# Autodesk Inventor assembly: Assembly2
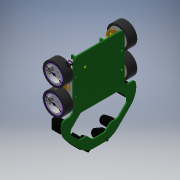
[picture p0: Inventor's stored thumbnail of the model, 180x180]
Saved by Autodesk Inventor 2016 (Build 200138000, 138)
## iProperties
Created: 2017-05-26
Part Number: Assembly2
Material: Ogólny
Document SubType Name: Assembly
Designer: Karol
Author: Karol
## Documents named in this file (32)
- D:\Git\MicromouseDixi\hardware\models\Dixi.iam
- D:\Git\MicromouseDixi\hardware\models\wheel.ipt
- D:\Git\MicromouseDixi\hardware\models\togh.ipt
- D:\Git\MicromouseDixi\hardware\models\bolt.ipt
- D:\Git\MicromouseDixi\hardware\models\magnet.ipt
- D:\Git\MicromouseDixi\hardware\models\mainpcb.ipt
- D:\Git\MicromouseDixi\hardware\models\motor.ipt
- D:\Git\MicromouseDixi\hardware\models\top_mount.ipt
- D:\Git\MicromouseDixi\hardware\models\XSM_0203_03_1.ipt
- D:\Git\MicromouseDixi\hardware\models\XFM_020406_03_233.ipt
- D:\Git\MicromouseDixi\hardware\models\enc_pcb.ipt
- D:\Git\MicromouseDixi\hardware\models\tyre.ipt
- D:\Git\MicromouseDixi\hardware\models\Dixi\Design Accelerator\Spur Gears4.iam
- D:\Git\MicromouseDixi\hardware\models\Dixi\Design Accelerator\Spur Gears3.iam
- D:\Git\MicromouseDixi\hardware\models\magnet_holder.ipt
- D:\Git\MicromouseDixi\hardware\models\tssop14.iam
- D:\Git\MicromouseDixi\hardware\models\led_mount.ipt
- D:\Git\MicromouseDixi\hardware\models\bolt_MIR.ipt
- D:\Git\MicromouseDixi\hardware\models\wheel_MIR.ipt
- D:\Git\MicromouseDixi\hardware\models\magnet_MIR.ipt
- D:\Git\MicromouseDixi\hardware\models\togh_MIR.ipt
- D:\Git\MicromouseDixi\hardware\models\motor_MIR.ipt
- D:\Git\MicromouseDixi\hardware\models\top_mount_MIR.ipt
- D:\Git\MicromouseDixi\hardware\models\XSM_0203_03_1_MIR.ipt
- D:\Git\MicromouseDixi\hardware\models\XFM_020406_03_233_MIR.ipt
- D:\Git\MicromouseDixi\hardware\models\enc_pcb_MIR.ipt
- D:\Git\MicromouseDixi\hardware\models\tyre_MIR.ipt
- D:\Git\MicromouseDixi\hardware\models\Dixi\Design Accelerator\Spur Gears4_MIR.iam
- D:\Git\MicromouseDixi\hardware\models\Dixi\Design Accelerator\Spur Gears3_MIR.iam
- D:\Git\MicromouseDixi\hardware\models\magnet_holder_MIR.ipt
- D:\Git\MicromouseDixi\hardware\models\tssop14_MIR.iam
- D:\Git\MicromouseDixi\hardware\models\led_mount_MIR.ipt
## Components (47 placed, 30 different names)
1. mainpcb:1 — Rotational:1, Rigid:47, Mate:1, Mate:2, Rigid:54
2. bolt:3 — Rigid:15, Rigid:45, Rotational:2
3. bolt:4 — Rigid:14, Rigid:46, Rigid:51, Rigid:52
4. wheel:3 — Rigid:15, Rigid:50
5. wheel:4 — Rigid:14, Rigid:49
6. magnet:4 — Rigid:53
7. togh:2 — Rigid:39, Rigid:40, Rigid:41, Rigid:44, Rotational:1, Rigid:47
8. motor:1 — Rigid:39, Rotational:3
9. top_mount:1 — Rigid:40
10. XSM_0203_03_1:1 — Rigid:42, Rigid:45
11. XFM_020406_03_233:1 — Rigid:41, Rigid:42
12. XSM_0203_03_1:2 — Rigid:46
13. XFM_020406_03_233:2 — Rigid:44
14. enc_pcb:1 — Planar:1, Rigid:54
15. tyre:1 — Rigid:49
16. tyre:2 — Rigid:50
17. Spur Gears:2 [sub-assembly] — Rigid:51
18. Spur Gears:7 [sub-assembly] — Rotational:2
19. Spur Gears:8 [sub-assembly] — Rotational:3
20. magnet_holder:1 — Rigid:52, Rigid:53
21. tssop14:1 [sub-assembly] — Planar:1
22. led_mount:1
23. led_mount:2
24. led_mount:3
25. bolt_MIR:1 — Rigid:55, Rigid:59, Rotational:4
26. bolt_MIR:2 — Rigid:56, Rigid:62, Rigid:67, Rigid:69
27. wheel_MIR:1 — Rigid:55, Rigid:66
28. wheel_MIR:2 — Rigid:56, Rigid:65
29. magnet_MIR:1 — Rigid:68
30. togh_MIR:1 — Rigid:57, Rigid:58, Rigid:60, Rigid:63
31. motor_MIR:1 — Rigid:57
32. top_mount_MIR:1 — Rigid:58
33. XSM_0203_03_1_MIR:1 — Rigid:59, Rigid:61
34. XFM_020406_03_233_MIR:1 — Rigid:60, Rigid:61
35. XSM_0203_03_1_MIR:2 — Rigid:62, Rigid:64
36. XFM_020406_03_233_MIR:2 — Rigid:63, Rigid:64
37. enc_pcb_MIR:1 — Planar:2
38. tyre_MIR:1 — Rigid:65
39. tyre_MIR:2 — Rigid:66
40. Spur Gears4_MIR:1 [sub-assembly] — Rigid:67
41. Spur Gears4_MIR:2 [sub-assembly] — Rotational:4
42. Spur Gears3_MIR:1 [sub-assembly]
43. magnet_holder_MIR:1 — Rigid:68, Rigid:69
44. tssop14_MIR:1 [sub-assembly] — Planar:2
45. led_mount_MIR:1
46. led_mount_MIR:2
47. led_mount_MIR:3
## Relationships (40: WeldJoint 32, RevoluteJoint 4, Mate 2, PlanarJoint 2)
- Rigid:14 [WeldJoint] (-1.8 mm): bolt:4 ↔ wheel:4
- Rigid:15 [WeldJoint] (-1.8 mm): bolt:3 ↔ wheel:3
- Rigid:39 [WeldJoint]: togh:2 ↔ motor:1
- Rigid:40 [WeldJoint]: togh:2 ↔ top_mount:1
- Rigid:41 [WeldJoint]: togh:2 ↔ XFM_020406_03_233:1
- Rigid:42 [WeldJoint] (-1.5 mm): XSM_0203_03_1:1 ↔ XFM_020406_03_233:1
- [WeldJoint]: XSM_0203_03_1:2 ↔ XFM_020406_03_233:2
- Rigid:44 [WeldJoint] (1 mm): togh:2 ↔ XFM_020406_03_233:2
- Rigid:45 [WeldJoint] (1.5 mm): bolt:3 ↔ XSM_0203_03_1:1
- Rigid:46 [WeldJoint]: bolt:4 ↔ XSM_0203_03_1:2
- Rotational:1 [RevoluteJoint]: mainpcb:1 ↔ togh:2
- Rigid:47 [WeldJoint]: mainpcb:1 ↔ togh:2
- Rigid:49 [WeldJoint]: wheel:4 ↔ tyre:1
- Rigid:50 [WeldJoint]: wheel:3 ↔ tyre:2
- Mate:1: mainpcb:1
- Mate:2: mainpcb:1
- Rotational:2 [RevoluteJoint] (1.5 mm): bolt:3 ↔ Spur Gears:7
- Rigid:51 [WeldJoint] (1.5 mm): bolt:4 ↔ Spur Gears:2
- Rotational:3 [RevoluteJoint] (-3.7 mm): motor:1 ↔ Spur Gears:8
- Rigid:52 [WeldJoint]: bolt:4 ↔ magnet_holder:1
- Rigid:53 [WeldJoint]: magnet:4 ↔ magnet_holder:1
- Planar:1: enc_pcb:1 ↔ tssop14:1
- Rigid:54 [WeldJoint]: mainpcb:1 ↔ enc_pcb:1
- Rigid:55 [WeldJoint] (-1.8 mm): bolt_MIR:1 ↔ wheel_MIR:1
- Rigid:56 [WeldJoint] (-1.8 mm): bolt_MIR:2 ↔ wheel_MIR:2
- Rigid:57 [WeldJoint]: togh_MIR:1 ↔ motor_MIR:1
- Rigid:58 [WeldJoint]: togh_MIR:1 ↔ top_mount_MIR:1
- Rigid:59 [WeldJoint] (1.5 mm): bolt_MIR:1 ↔ XSM_0203_03_1_MIR:1
- Rigid:60 [WeldJoint]: togh_MIR:1 ↔ XFM_020406_03_233_MIR:1
- Rigid:61 [WeldJoint] (-1.5 mm): XSM_0203_03_1_MIR:1 ↔ XFM_020406_03_233_MIR:1
- Rigid:62 [WeldJoint]: bolt_MIR:2 ↔ XSM_0203_03_1_MIR:2
- Rigid:63 [WeldJoint] (1 mm): togh_MIR:1 ↔ XFM_020406_03_233_MIR:2
- Rigid:64 [WeldJoint]: XSM_0203_03_1_MIR:2 ↔ XFM_020406_03_233_MIR:2
- Rigid:65 [WeldJoint]: wheel_MIR:2 ↔ tyre_MIR:1
- Rigid:66 [WeldJoint]: wheel_MIR:1 ↔ tyre_MIR:2
- Rigid:67 [WeldJoint] (1.5 mm): bolt_MIR:2 ↔ Spur Gears4_MIR:1
- Rotational:4 [RevoluteJoint] (-1.5 mm): bolt_MIR:1 ↔ Spur Gears4_MIR:2
- Rigid:68 [WeldJoint]: magnet_MIR:1 ↔ magnet_holder_MIR:1
- Rigid:69 [WeldJoint]: bolt_MIR:2 ↔ magnet_holder_MIR:1
- Planar:2: enc_pcb_MIR:1 ↔ tssop14_MIR:1
## Named parameters: d111_d4 = -1.8 mm, d112_d5 = 0.127925 deg, d113_d6 = -1.8 mm, d114_d7 = -6.839272 deg, d234_d233 = 0 mm
